# Autodesk Inventor assembly: Frame
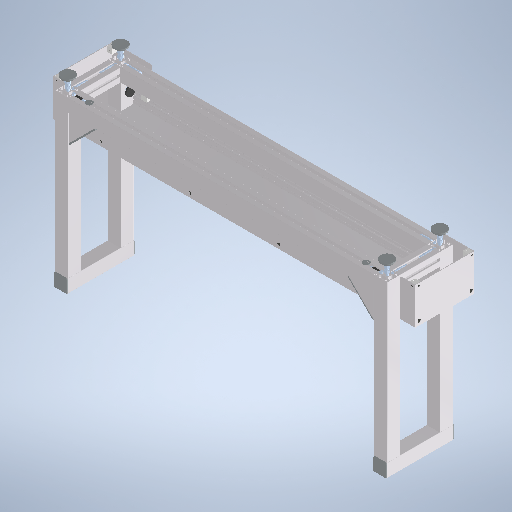
[picture p0: Inventor's stored thumbnail of the model, 512x512]
Saved by Autodesk Inventor 2025 (Build 290162010, 162A)
## iProperties
Created: 2025-01-18
Part Number: Frame
Document SubType Name: Assembly
Designer: Admin
Mass: 13411.7 g
Surface Area: 37015.5 cm^2
Volume: 4609.9 cm^3
Density: 2.90933 g/cm^3
Author: Admin
## Documents named in this file (34)
- C:\Users\Admin\GIT\HDVKBM\CAD\Krandemonstrator\Frame.iam
- C:\Users\Admin\GIT\HDVKBM\CAD\Krandemonstrator\item_61193_profil-x-8-40x40-2no180-_930_high\item_61193_profil-x-8-40x40-2no180-_930_high.ipt
- C:\Users\Admin\GIT\HDVKBM\CAD\Krandemonstrator\item_49291_profil-x-8-40x40-leicht-_120_high\item_49291_profil-x-8-40x40-leicht-_120_high.ipt
- C:\Users\Admin\GIT\HDVKBM\CAD\Krandemonstrator\item_49288_profil-x-8-40x40-4no-lei_200_high\item_49288_profil-x-8-40x40-4no-lei_200_high.ipt
- C:\Users\Admin\GIT\HDVKBM\CAD\Krandemonstrator\item_49288_profil-x-8-40x40-4no-lei_475_high\item_49288_profil-x-8-40x40-4no-lei_475_high.ipt
- C:\Users\Admin\GIT\HDVKBM\CAD\Krandemonstrator\item_67284_automatik-verbindungssat__high\item_67284_automatik-verbindungssat__high.ipt
- C:\Users\Admin\GIT\HDVKBM\CAD\Krandemonstrator\item_63697_stellfuss-d40-m8x60-grau_35_0_high\item_63697_stellfuss-d40-m8x60-grau_35_0_high.ipt
- C:\Users\Admin\GIT\HDVKBM\CAD\Krandemonstrator\item_62716_abdeckkappe-8-40x40-grau__high\item_62716_abdeckkappe-8-40x40-grau__high.ipt
- C:\Users\Admin\GIT\HDVKBM\CAD\Krandemonstrator\item_48996_automatik-verbindungssat__high\item_48996_automatik-verbindungssat__high.ipt
- C:\Users\Admin\GIT\HDVKBM\CAD\Krandemonstrator\item_41123_winkel-8-80x80-zn-weissa__high\item_41123_winkel-8-80x80-zn-weissa__high.ipt
- C:\Users\Admin\GIT\HDVKBM\CAD\Krandemonstrator\item_2618_nutenstein-8-st-m8-verzi__high\item_2618_nutenstein-8-st-m8-verzi__high.ipt
- C:\Users\Admin\GIT\HDVKBM\CAD\Krandemonstrator\item_62758_winkel-abdeckkappe-8-80x__high\item_62758_winkel-abdeckkappe-8-80x__high.ipt
- C:\Users\Admin\GIT\HDVKBM\CAD\Krandemonstrator\item_43452_stellfuss-d30-m6x45-schw_20_0_high\item_43452_stellfuss-d30-m6x45-schw_20_0_high.ipt
- C:\Users\Admin\GIT\HDVKBM\CAD\Krandemonstrator\item_2623_nutenstein-8-st-m6-verzi__high\item_2623_nutenstein-8-st-m6-verzi__high.ipt
- C:\Users\Admin\GIT\HDVKBM\CAD\Krandemonstrator\item_42005_nutenstein-8-st-m5-verzi__high\item_42005_nutenstein-8-st-m5-verzi__high.ipt
- C:\Users\Admin\GIT\HDVKBM\CAD\Krandemonstrator\item_67777_winkel-5-20-weissalumini__high\item_67777_winkel-5-20-weissalumini__high.ipt
- C:\Users\Admin\GIT\HDVKBM\CAD\Krandemonstrator\item_68092_befestigungssatz-5-2-4mm_2_high\item_68092_befestigungssatz-5-2-4mm_2_high.ipt
- C:\Users\Admin\GIT\HDVKBM\CAD\Krandemonstrator\item_47308_blech-al-2mm-naturfarben_1100_180_high\item_47308_blech-al-2mm-naturfarben_1100_180_high.ipt
- C:\Users\Admin\GIT\HDVKBM\CAD\Krandemonstrator\item_37006_nutenstein-5-st-m4-verzi__high\item_37006_nutenstein-5-st-m4-verzi__high.ipt
- C:\Users\Admin\GIT\HDVKBM\CAD\Krandemonstrator\item_47308_blech-al-2mm-naturfarben_110_1100_high\item_47308_blech-al-2mm-naturfarben_110_1100_high.ipt
- C:\Users\Admin\GIT\HDVKBM\CAD\Krandemonstrator\item_37003_profil-5-20x20-natur-370_1096_high\item_37003_profil-5-20x20-natur-370_1096_high.ipt
- C:\Users\Admin\GIT\HDVKBM\CAD\Krandemonstrator\item_43774_profil-5-20x20-1n-natur-_1096_high\item_43774_profil-5-20x20-1n-natur-_1096_high.ipt
- C:\Users\Admin\GIT\HDVKBM\CAD\Krandemonstrator\item_47308_blech-al-2mm-naturfarben_178_110_high\item_47308_blech-al-2mm-naturfarben_178_110_high.ipt
- C:\Users\Admin\GIT\HDVKBM\CAD\Krandemonstrator\item_47308_blech-al-2mm-naturfarben_120_90_high\item_47308_blech-al-2mm-naturfarben_120_90_high.ipt
- C:\Users\Admin\GIT\HDVKBM\CAD\Krandemonstrator\Frameblock.ipt
- C:\Users\Admin\GIT\HDVKBM\CAD\Krandemonstrator\item_47308_blech-al-2mm-naturfarben_120_90_high\item_47308_blech-al-2mm-naturfarben_120_90_highLH.ipt
- C:\Users\Admin\GIT\HDVKBM\CAD\Krandemonstrator\item_61196_profil-x-8-40x40-3no-lei_930_high\item_61196_profil-x-8-40x40-3no-lei_930_high.ipt
- C:\Users\Admin\Documents\Inventor\Content Center Files\R2025\de-DE\ISO 10642(2)\ISO 10642  - M3  x  8.ipt
- C:\Users\Admin\Documents\Inventor\Content Center Files\R2025\de-DE\ISO 10642(2)\ISO 10642  - M4  x  20.ipt
- C:\Users\Admin\Documents\Inventor\Content Center Files\R2025\de-DE\ISO 10642(2)\ISO 10642  - M4  x  8.ipt
- C:\Users\Admin\Documents\Inventor\Content Center Files\R2025\de-DE\ISO 10642(2)\ISO 10642  - M5  x  10.ipt
- C:\Users\Admin\Documents\Inventor\Content Center Files\R2025\de-DE\ISO 10642(2)\ISO 10642  - M5  x  12.ipt
- C:\Users\Admin\Documents\Inventor\Content Center Files\R2025\de-DE\ISO 10642(2)\ISO 10642  - M5  x  16.ipt
- C:\Users\Admin\Documents\Inventor\Content Center Files\R2025\de-DE\ISO 4762(1)\DIN EN ISO 4762 - M8 x 16.ipt
## Components (126 placed, 33 different names)
1. item_61193_profil-x-8-40x40-2no180-_930_high:1 — Starr:12, Starr:13, Starr:14
2. item_61196_profil-x-8-40x40-3no-lei_930_high:1 — Starr:17, Starr:27, Planar:1, Planar:2, Starr:47, Starr:48, Planar:68, Verschiebbar:70
3. item_49291_profil-x-8-40x40-leicht-_120_high:1 — Starr:7, Starr:8, Starr:9
4. item_49291_profil-x-8-40x40-leicht-_120_high:2 — Starr:24, Starr:25, Starr:26
5. item_49288_profil-x-8-40x40-4no-lei_200_high:1 — Starr:18, Starr:19, Starr:21, Starr:23
6. item_49288_profil-x-8-40x40-4no-lei_200_high:2 — Starr:2, Starr:4, Starr:5, Starr:6
7. item_49288_profil-x-8-40x40-4no-lei_475_high:1 — Starr:20, Starr:21, Starr:28, Starr:41, Verschiebbar:6
8. item_49288_profil-x-8-40x40-4no-lei_475_high:2 — Starr:22, Starr:23, Starr:25, Starr:27, Starr:29, Verschiebbar:2, Verschiebbar:4
9. item_49288_profil-x-8-40x40-4no-lei_475_high:3 — Starr:3, Starr:4, Starr:11, Starr:17, Verschiebbar:1, Verschiebbar:3, Planar:71
10. item_49288_profil-x-8-40x40-4no-lei_475_high:4 — Starr:1, Starr:2, Starr:9, Starr:10, Starr:14, Starr:43, Verschiebbar:5
11. item_67284_automatik-verbindungssat__high:1 — Starr:1
12. item_67284_automatik-verbindungssat__high:2 — Starr:20
13. item_67284_automatik-verbindungssat__high:3 — Starr:3
14. item_67284_automatik-verbindungssat__high:11 — Starr:22
15. item_67284_automatik-verbindungssat__high:4 — Starr:24
16. item_67284_automatik-verbindungssat__high:12 — Starr:26
17. item_67284_automatik-verbindungssat__high:5 — Starr:12
18. item_67284_automatik-verbindungssat__high:6 — Starr:13
19. item_67284_automatik-verbindungssat__high:7 — Starr:8
20. item_67284_automatik-verbindungssat__high:8 — Starr:7
21. item_48996_automatik-verbindungssat__high:1 — Starr:47
22. item_48996_automatik-verbindungssat__high:2 — Starr:48
23. item_63697_stellfuss-d40-m8x60-grau_35_0_high:1 — Starr:10
24. item_63697_stellfuss-d40-m8x60-grau_35_0_high:2 — Starr:11
25. item_63697_stellfuss-d40-m8x60-grau_35_0_high:3 — Starr:28
26. item_63697_stellfuss-d40-m8x60-grau_35_0_high:4 — Starr:29
27. item_62716_abdeckkappe-8-40x40-grau__high:1 — Starr:5
28. item_62716_abdeckkappe-8-40x40-grau__high:2 — Starr:6
29. item_62716_abdeckkappe-8-40x40-grau__high:3 — Starr:18
30. item_62716_abdeckkappe-8-40x40-grau__high:4 — Starr:19
31. item_41123_winkel-8-80x80-zn-weissa__high:1 — Verschiebbar:2, Planar:2, Starr:38
32. item_41123_winkel-8-80x80-zn-weissa__high:2 — Verschiebbar:1, Planar:1, Starr:39
33. item_2618_nutenstein-8-st-m8-verzi__high:5
34. item_2618_nutenstein-8-st-m8-verzi__high:3
35. item_2618_nutenstein-8-st-m8-verzi__high:2
36. item_2618_nutenstein-8-st-m8-verzi__high:6
37. item_2618_nutenstein-8-st-m8-verzi__high:4
38. item_2618_nutenstein-8-st-m8-verzi__high:8
39. item_2618_nutenstein-8-st-m8-verzi__high:1
40. item_2618_nutenstein-8-st-m8-verzi__high:7
41. DIN EN ISO 4762 M8 x 16:1
42. DIN EN ISO 4762 M8 x 16:2
43. DIN EN ISO 4762 M8 x 16:3
44. DIN EN ISO 4762 M8 x 16:4
45. DIN EN ISO 4762 M8 x 16:5
46. DIN EN ISO 4762 M8 x 16:6
47. DIN EN ISO 4762 M8 x 16:7
48. DIN EN ISO 4762 M8 x 16:8
49. item_62758_winkel-abdeckkappe-8-80x__high:1 — Starr:38
50. item_62758_winkel-abdeckkappe-8-80x__high:2 — Starr:39
51. item_2623_nutenstein-8-st-m6-verzi__high:2 — Starr:42, Starr:43
52. item_2623_nutenstein-8-st-m6-verzi__high:1 — Starr:40, Starr:41
53. item_43452_stellfuss-d30-m6x45-schw_20_0_high:1 — Starr:40
54. item_43452_stellfuss-d30-m6x45-schw_20_0_high:2 — Starr:42
55. Frameblock:1 — Starr:73, Starr:84
56. Frameblock:2 — Starr:74, Starr:83
57. Frameblock:3 — Starr:75
58. Frameblock:4 — Starr:76, Starr:82
59. Frameblock:5 — Starr:78
60. Frameblock:6 — Starr:77, Starr:81
61. Frameblock:7 — Starr:79
62. Frameblock:8 — Starr:80
63. item_37006_nutenstein-5-st-m4-verzi__high:1 — Starr:61
64. item_37006_nutenstein-5-st-m4-verzi__high:2 — Starr:63
65. item_37006_nutenstein-5-st-m4-verzi__high:3 — Starr:62
66. item_37006_nutenstein-5-st-m4-verzi__high:4 — Starr:60
67. item_37006_nutenstein-5-st-m4-verzi__high:5 — Starr:81
68. item_37006_nutenstein-5-st-m4-verzi__high:6 — Starr:84
69. item_37006_nutenstein-5-st-m4-verzi__high:7 — Starr:82
70. item_37006_nutenstein-5-st-m4-verzi__high:8 — Starr:83
71. item_37006_nutenstein-5-st-m4-verzi__high:9
72. item_37006_nutenstein-5-st-m4-verzi__high:10
73. item_37006_nutenstein-5-st-m4-verzi__high:11
74. item_37006_nutenstein-5-st-m4-verzi__high:12
75. item_42005_nutenstein-8-st-m5-verzi__high:1 — Starr:45
76. item_42005_nutenstein-8-st-m5-verzi__high:2 — Starr:44
77. item_42005_nutenstein-8-st-m5-verzi__high:3 — Starr:52
78. item_42005_nutenstein-8-st-m5-verzi__high:4 — Starr:53
79. item_43774_profil-5-20x20-1n-natur-_1096_high:1 — Planar:73, Planar:76
80. item_37003_profil-5-20x20-natur-370_1096_high:1
81. item_47308_blech-al-2mm-naturfarben_110_1100_high:1 — Starr:64, Starr:65, Starr:66, Starr:67, Planar:71, Starr:68, Verschiebbar:70, Starr:69, Starr:70
82. item_47308_blech-al-2mm-naturfarben_178_110_high:1 — Starr:69, Starr:71, Starr:80
83. item_47308_blech-al-2mm-naturfarben_178_110_high:2 — Starr:70, Starr:72, Starr:79
84. item_47308_blech-al-2mm-naturfarben_120_90_highLH:1 — Starr:72, Starr:76, Starr:77, Starr:78
85. item_47308_blech-al-2mm-naturfarben_120_90_high:2 — Starr:71, Starr:73, Starr:74, Starr:75
86. item_47308_blech-al-2mm-naturfarben_1100_180_high:1 — Planar:68, Starr:68, Planar:76
87. item_67777_winkel-5-20-weissalumini__high:1 — Starr:44, Starr:49, Verschiebbar:6, Planar:73
88. item_67777_winkel-5-20-weissalumini__high:2 — Starr:45, Starr:46, Verschiebbar:5
89. item_67777_winkel-5-20-weissalumini__high:3 — Starr:50, Starr:53, Verschiebbar:4
90. item_67777_winkel-5-20-weissalumini__high:4 — Starr:51, Starr:52, Verschiebbar:3
91. item_68092_befestigungssatz-5-2-4mm_2_high:1 — Starr:49
92. item_68092_befestigungssatz-5-2-4mm_2_high:2 — Starr:46
93. item_68092_befestigungssatz-5-2-4mm_2_high:3 — Starr:50
94. item_68092_befestigungssatz-5-2-4mm_2_high:4 — Starr:51
95. DIN EN ISO 10642 M3  x  8:1
96. DIN EN ISO 10642 M3  x  8:2
97. DIN EN ISO 10642 M3  x  8:3
98. DIN EN ISO 10642 M4  x  20:1
99. DIN EN ISO 10642 M3  x  8:4
100. DIN EN ISO 10642 M3  x  8:5
101. DIN EN ISO 10642 M3  x  8:6
102. DIN EN ISO 10642 M4  x  20:2
103. DIN EN ISO 10642 M3  x  8:7
104. DIN EN ISO 10642 M3  x  8:8
105. DIN EN ISO 10642 M3  x  8:9
106. DIN EN ISO 10642 M3  x  8:10
107. DIN EN ISO 10642 M3  x  8:11
108. DIN EN ISO 10642 M3  x  8:12
109. DIN EN ISO 10642 M4  x  20:3
110. DIN EN ISO 10642 M4  x  20:4
111. DIN EN ISO 10642 M4  x  8:1
112. DIN EN ISO 10642 M4  x  8:2
113. DIN EN ISO 10642 M4  x  8:3
114. DIN EN ISO 10642 M4  x  8:4
115. DIN EN ISO 10642 M5  x  10:1
116. DIN EN ISO 10642 M5  x  10:2
117. DIN EN ISO 10642 M5  x  10:3
118. DIN EN ISO 10642 M5  x  10:4
119. DIN EN ISO 10642 M4  x  8:5 — Starr:60, Starr:67
120. DIN EN ISO 10642 M4  x  8:6 — Starr:62, Starr:64
121. DIN EN ISO 10642 M4  x  8:7 — Starr:61, Starr:66
122. DIN EN ISO 10642 M4  x  8:8 — Starr:63, Starr:65
123. DIN EN ISO 10642 M5  x  12:1
124. DIN EN ISO 10642 M5  x  12:2
125. DIN EN ISO 10642 M5  x  16:1
126. DIN EN ISO 10642 M5  x  16:2
## Relationships (138: WeldJoint 84, Mate 24, PlanarJoint 14, Insert 8, TranslationJoint 8)
- Starr:1 [WeldJoint]: item_49288_profil-x-8-40x40-4no-lei_475_high:4 ↔ item_67284_automatik-verbindungssat__high:1
- Starr:2 [WeldJoint]: item_49288_profil-x-8-40x40-4no-lei_200_high:2 ↔ item_49288_profil-x-8-40x40-4no-lei_475_high:4
- Starr:3 [WeldJoint]: item_49288_profil-x-8-40x40-4no-lei_475_high:3 ↔ item_67284_automatik-verbindungssat__high:3
- Starr:4 [WeldJoint]: item_49288_profil-x-8-40x40-4no-lei_200_high:2 ↔ item_49288_profil-x-8-40x40-4no-lei_475_high:3
- Starr:5 [WeldJoint]: item_49288_profil-x-8-40x40-4no-lei_200_high:2 ↔ item_62716_abdeckkappe-8-40x40-grau__high:1
- Starr:6 [WeldJoint]: item_49288_profil-x-8-40x40-4no-lei_200_high:2 ↔ item_62716_abdeckkappe-8-40x40-grau__high:2
- Starr:7 [WeldJoint]: item_49291_profil-x-8-40x40-leicht-_120_high:1 ↔ item_67284_automatik-verbindungssat__high:8
- Starr:8 [WeldJoint]: item_49291_profil-x-8-40x40-leicht-_120_high:1 ↔ item_67284_automatik-verbindungssat__high:7
- Starr:9 [WeldJoint]: item_49291_profil-x-8-40x40-leicht-_120_high:1 ↔ item_49288_profil-x-8-40x40-4no-lei_475_high:4
- Starr:10 [WeldJoint]: item_49288_profil-x-8-40x40-4no-lei_475_high:4 ↔ item_63697_stellfuss-d40-m8x60-grau_35_0_high:1
- Starr:11 [WeldJoint]: item_49288_profil-x-8-40x40-4no-lei_475_high:3 ↔ item_63697_stellfuss-d40-m8x60-grau_35_0_high:2
- Starr:12 [WeldJoint]: item_61193_profil-x-8-40x40-2no180-_930_high:1 ↔ item_67284_automatik-verbindungssat__high:5
- Starr:13 [WeldJoint]: item_61193_profil-x-8-40x40-2no180-_930_high:1 ↔ item_67284_automatik-verbindungssat__high:6
- Starr:14 [WeldJoint]: item_61193_profil-x-8-40x40-2no180-_930_high:1 ↔ item_49288_profil-x-8-40x40-4no-lei_475_high:4
- Starr:17 [WeldJoint]: item_61196_profil-x-8-40x40-3no-lei_930_high:1 ↔ item_49288_profil-x-8-40x40-4no-lei_475_high:3
- Starr:18 [WeldJoint]: item_49288_profil-x-8-40x40-4no-lei_200_high:1 ↔ item_62716_abdeckkappe-8-40x40-grau__high:3
- Starr:19 [WeldJoint]: item_49288_profil-x-8-40x40-4no-lei_200_high:1 ↔ item_62716_abdeckkappe-8-40x40-grau__high:4
- Starr:20 [WeldJoint]: item_49288_profil-x-8-40x40-4no-lei_475_high:1 ↔ item_67284_automatik-verbindungssat__high:2
- Starr:21 [WeldJoint]: item_49288_profil-x-8-40x40-4no-lei_200_high:1 ↔ item_49288_profil-x-8-40x40-4no-lei_475_high:1
- Starr:22 [WeldJoint]: item_49288_profil-x-8-40x40-4no-lei_475_high:2 ↔ item_67284_automatik-verbindungssat__high:11
- Starr:23 [WeldJoint]: item_49288_profil-x-8-40x40-4no-lei_200_high:1 ↔ item_49288_profil-x-8-40x40-4no-lei_475_high:2
- Starr:24 [WeldJoint]: item_49291_profil-x-8-40x40-leicht-_120_high:2 ↔ item_67284_automatik-verbindungssat__high:4
- Starr:25 [WeldJoint]: item_49291_profil-x-8-40x40-leicht-_120_high:2 ↔ item_49288_profil-x-8-40x40-4no-lei_475_high:2
- Starr:26 [WeldJoint]: item_49291_profil-x-8-40x40-leicht-_120_high:2 ↔ item_67284_automatik-verbindungssat__high:12
- Starr:27 [WeldJoint]: item_61196_profil-x-8-40x40-3no-lei_930_high:1 ↔ item_49288_profil-x-8-40x40-4no-lei_475_high:2
- Starr:28 [WeldJoint]: item_49288_profil-x-8-40x40-4no-lei_475_high:1 ↔ item_63697_stellfuss-d40-m8x60-grau_35_0_high:3
- Starr:29 [WeldJoint]: item_49288_profil-x-8-40x40-4no-lei_475_high:2 ↔ item_63697_stellfuss-d40-m8x60-grau_35_0_high:4
- [Insert]: item_41123_winkel-8-80x80-zn-weissa__high:2 ↔ DIN EN ISO 4762 M8 x 16:1
- [Insert]: item_41123_winkel-8-80x80-zn-weissa__high:2 ↔ DIN EN ISO 4762 M8 x 16:2
- [Insert]: item_41123_winkel-8-80x80-zn-weissa__high:1 ↔ DIN EN ISO 4762 M8 x 16:3
- [Insert]: item_41123_winkel-8-80x80-zn-weissa__high:1 ↔ DIN EN ISO 4762 M8 x 16:4
- [Insert]: item_41123_winkel-8-80x80-zn-weissa__high:2 ↔ DIN EN ISO 4762 M8 x 16:5
- [Insert]: item_41123_winkel-8-80x80-zn-weissa__high:2 ↔ DIN EN ISO 4762 M8 x 16:6
- [Insert]: item_41123_winkel-8-80x80-zn-weissa__high:1 ↔ DIN EN ISO 4762 M8 x 16:7
- [Insert]: item_41123_winkel-8-80x80-zn-weissa__high:1 ↔ DIN EN ISO 4762 M8 x 16:8
- [WeldJoint]: item_2618_nutenstein-8-st-m8-verzi__high:6 ↔ DIN EN ISO 4762 M8 x 16:6
- [WeldJoint]: item_2618_nutenstein-8-st-m8-verzi__high:2 ↔ DIN EN ISO 4762 M8 x 16:5
- [WeldJoint]: item_2618_nutenstein-8-st-m8-verzi__high:4 ↔ DIN EN ISO 4762 M8 x 16:8
- [WeldJoint]: item_2618_nutenstein-8-st-m8-verzi__high:8 ↔ DIN EN ISO 4762 M8 x 16:7
- [WeldJoint]: item_2618_nutenstein-8-st-m8-verzi__high:1 ↔ DIN EN ISO 4762 M8 x 16:4
- [WeldJoint]: item_2618_nutenstein-8-st-m8-verzi__high:7 ↔ DIN EN ISO 4762 M8 x 16:3
- [WeldJoint]: item_2618_nutenstein-8-st-m8-verzi__high:3 ↔ DIN EN ISO 4762 M8 x 16:2
- [WeldJoint]: item_2618_nutenstein-8-st-m8-verzi__high:5 ↔ DIN EN ISO 4762 M8 x 16:1
- Verschiebbar:1 [TranslationJoint]: item_49288_profil-x-8-40x40-4no-lei_475_high:3 ↔ item_41123_winkel-8-80x80-zn-weissa__high:2
- Planar:1: item_61196_profil-x-8-40x40-3no-lei_930_high:1 ↔ item_41123_winkel-8-80x80-zn-weissa__high:2
- Verschiebbar:2 [TranslationJoint]: item_49288_profil-x-8-40x40-4no-lei_475_high:2 ↔ item_41123_winkel-8-80x80-zn-weissa__high:1
- Planar:2: item_61196_profil-x-8-40x40-3no-lei_930_high:1 ↔ item_41123_winkel-8-80x80-zn-weissa__high:1
- Starr:38 [WeldJoint]: item_41123_winkel-8-80x80-zn-weissa__high:1 ↔ item_62758_winkel-abdeckkappe-8-80x__high:1
- Starr:39 [WeldJoint]: item_41123_winkel-8-80x80-zn-weissa__high:2 ↔ item_62758_winkel-abdeckkappe-8-80x__high:2
- Starr:40 [WeldJoint]: item_2623_nutenstein-8-st-m6-verzi__high:1 ↔ item_43452_stellfuss-d30-m6x45-schw_20_0_high:1
- Starr:41 [WeldJoint] (-60 mm): item_49288_profil-x-8-40x40-4no-lei_475_high:1 ↔ item_2623_nutenstein-8-st-m6-verzi__high:1
- Starr:42 [WeldJoint]: item_2623_nutenstein-8-st-m6-verzi__high:2 ↔ item_43452_stellfuss-d30-m6x45-schw_20_0_high:2
- Starr:43 [WeldJoint] (-60 mm): item_49288_profil-x-8-40x40-4no-lei_475_high:4 ↔ item_2623_nutenstein-8-st-m6-verzi__high:2
- Starr:44 [WeldJoint] (-5 mm): item_42005_nutenstein-8-st-m5-verzi__high:2 ↔ item_67777_winkel-5-20-weissalumini__high:1
- Starr:45 [WeldJoint] (-5 mm): item_42005_nutenstein-8-st-m5-verzi__high:1 ↔ item_67777_winkel-5-20-weissalumini__high:2
- Starr:46 [WeldJoint]: item_67777_winkel-5-20-weissalumini__high:2 ↔ item_68092_befestigungssatz-5-2-4mm_2_high:2
- Starr:47 [WeldJoint]: item_61196_profil-x-8-40x40-3no-lei_930_high:1 ↔ item_48996_automatik-verbindungssat__high:1
- Starr:48 [WeldJoint]: item_61196_profil-x-8-40x40-3no-lei_930_high:1 ↔ item_48996_automatik-verbindungssat__high:2
- Starr:49 [WeldJoint]: item_67777_winkel-5-20-weissalumini__high:1 ↔ item_68092_befestigungssatz-5-2-4mm_2_high:1
- [Mate]: item_67777_winkel-5-20-weissalumini__high:1 ↔ DIN EN ISO 10642 M5  x  12:1
- [Mate]: item_67777_winkel-5-20-weissalumini__high:2 ↔ DIN EN ISO 10642 M5  x  12:2
- Starr:50 [WeldJoint]: item_67777_winkel-5-20-weissalumini__high:3 ↔ item_68092_befestigungssatz-5-2-4mm_2_high:3
- Starr:51 [WeldJoint]: item_67777_winkel-5-20-weissalumini__high:4 ↔ item_68092_befestigungssatz-5-2-4mm_2_high:4
- [Mate]: item_67777_winkel-5-20-weissalumini__high:3 ↔ DIN EN ISO 10642 M5  x  16:1
- [Mate]: item_67777_winkel-5-20-weissalumini__high:4 ↔ DIN EN ISO 10642 M5  x  16:2
- Starr:52 [WeldJoint] (-5 mm): item_42005_nutenstein-8-st-m5-verzi__high:3 ↔ item_67777_winkel-5-20-weissalumini__high:4
- Starr:53 [WeldJoint] (-5 mm): item_42005_nutenstein-8-st-m5-verzi__high:4 ↔ item_67777_winkel-5-20-weissalumini__high:3
- Verschiebbar:3 [TranslationJoint] (2 mm): item_49288_profil-x-8-40x40-4no-lei_475_high:3 ↔ item_67777_winkel-5-20-weissalumini__high:4
- Verschiebbar:4 [TranslationJoint]: item_49288_profil-x-8-40x40-4no-lei_475_high:2 ↔ item_67777_winkel-5-20-weissalumini__high:3
- [PlanarJoint]: item_37003_profil-5-20x20-natur-370_1096_high:1 ↔ item_67777_winkel-5-20-weissalumini__high:4
- [PlanarJoint]: item_37003_profil-5-20x20-natur-370_1096_high:1 ↔ item_67777_winkel-5-20-weissalumini__high:3
- Verschiebbar:5 [TranslationJoint]: item_49288_profil-x-8-40x40-4no-lei_475_high:4 ↔ item_67777_winkel-5-20-weissalumini__high:2
- Verschiebbar:6 [TranslationJoint]: item_49288_profil-x-8-40x40-4no-lei_475_high:1 ↔ item_67777_winkel-5-20-weissalumini__high:1
- [PlanarJoint]: item_37003_profil-5-20x20-natur-370_1096_high:1 ↔ item_47308_blech-al-2mm-naturfarben_1100_180_high:1
- Starr:60 [WeldJoint]: item_37006_nutenstein-5-st-m4-verzi__high:4 ↔ DIN EN ISO 10642 M4  x  8:5
- Starr:61 [WeldJoint]: item_37006_nutenstein-5-st-m4-verzi__high:1 ↔ DIN EN ISO 10642 M4  x  8:7
- Starr:62 [WeldJoint]: item_37006_nutenstein-5-st-m4-verzi__high:3 ↔ DIN EN ISO 10642 M4  x  8:6
- Starr:63 [WeldJoint]: item_37006_nutenstein-5-st-m4-verzi__high:2 ↔ DIN EN ISO 10642 M4  x  8:8
- Planar:68 (75 mm): item_61196_profil-x-8-40x40-3no-lei_930_high:1 ↔ item_47308_blech-al-2mm-naturfarben_1100_180_high:1
- Starr:64 [WeldJoint]: item_47308_blech-al-2mm-naturfarben_110_1100_high:1 ↔ DIN EN ISO 10642 M4  x  8:6
- Starr:65 [WeldJoint]: item_47308_blech-al-2mm-naturfarben_110_1100_high:1 ↔ DIN EN ISO 10642 M4  x  8:8
- Starr:66 [WeldJoint]: item_47308_blech-al-2mm-naturfarben_110_1100_high:1 ↔ DIN EN ISO 10642 M4  x  8:7
- Starr:67 [WeldJoint]: item_47308_blech-al-2mm-naturfarben_110_1100_high:1 ↔ DIN EN ISO 10642 M4  x  8:5
- [PlanarJoint]: item_37003_profil-5-20x20-natur-370_1096_high:1 ↔ item_47308_blech-al-2mm-naturfarben_110_1100_high:1
- [PlanarJoint]: item_37003_profil-5-20x20-natur-370_1096_high:1 ↔ item_47308_blech-al-2mm-naturfarben_110_1100_high:1
- [TranslationJoint]: item_37003_profil-5-20x20-natur-370_1096_high:1 ↔ item_47308_blech-al-2mm-naturfarben_110_1100_high:1
- Planar:71: item_49288_profil-x-8-40x40-4no-lei_475_high:3 ↔ item_47308_blech-al-2mm-naturfarben_110_1100_high:1
- Starr:68 [WeldJoint]: item_47308_blech-al-2mm-naturfarben_110_1100_high:1 ↔ item_47308_blech-al-2mm-naturfarben_1100_180_high:1
- Verschiebbar:70 [TranslationJoint]: item_61196_profil-x-8-40x40-3no-lei_930_high:1 ↔ item_47308_blech-al-2mm-naturfarben_110_1100_high:1
- [PlanarJoint]: item_43774_profil-5-20x20-1n-natur-_1096_high:1 ↔ item_47308_blech-al-2mm-naturfarben_1100_180_high:1
- Planar:73: item_43774_profil-5-20x20-1n-natur-_1096_high:1 ↔ item_67777_winkel-5-20-weissalumini__high:1
- [PlanarJoint]: item_43774_profil-5-20x20-1n-natur-_1096_high:1 ↔ item_67777_winkel-5-20-weissalumini__high:2
- [PlanarJoint]: item_49288_profil-x-8-40x40-4no-lei_475_high:4 ↔ item_43774_profil-5-20x20-1n-natur-_1096_high:1
- Planar:76 (-2 mm): item_43774_profil-5-20x20-1n-natur-_1096_high:1 ↔ item_47308_blech-al-2mm-naturfarben_1100_180_high:1
- Starr:69 [WeldJoint]: item_47308_blech-al-2mm-naturfarben_110_1100_high:1 ↔ item_47308_blech-al-2mm-naturfarben_178_110_high:1
- Starr:70 [WeldJoint]: item_47308_blech-al-2mm-naturfarben_110_1100_high:1 ↔ item_47308_blech-al-2mm-naturfarben_178_110_high:2
- Starr:71 [WeldJoint]: item_47308_blech-al-2mm-naturfarben_178_110_high:1 ↔ item_47308_blech-al-2mm-naturfarben_120_90_high:2
- Starr:72 [WeldJoint]: item_47308_blech-al-2mm-naturfarben_178_110_high:2 ↔ item_47308_blech-al-2mm-naturfarben_120_90_highLH:1
- [Mate]: item_47308_blech-al-2mm-naturfarben_178_110_high:1 ↔ DIN EN ISO 10642 M5  x  10:1
- [Mate]: item_47308_blech-al-2mm-naturfarben_178_110_high:1 ↔ DIN EN ISO 10642 M5  x  10:2
- [Mate]: item_47308_blech-al-2mm-naturfarben_178_110_high:2 ↔ DIN EN ISO 10642 M5  x  10:3
- [Mate]: item_47308_blech-al-2mm-naturfarben_178_110_high:2 ↔ DIN EN ISO 10642 M5  x  10:4
- Starr:73 [WeldJoint]: Frameblock:1 ↔ item_47308_blech-al-2mm-naturfarben_120_90_high:2
- Starr:74 [WeldJoint]: Frameblock:2 ↔ item_47308_blech-al-2mm-naturfarben_120_90_high:2
- Starr:75 [WeldJoint]: Frameblock:3 ↔ item_47308_blech-al-2mm-naturfarben_120_90_high:2
- Starr:76 [WeldJoint]: Frameblock:4 ↔ item_47308_blech-al-2mm-naturfarben_120_90_highLH:1
- Starr:77 [WeldJoint]: Frameblock:6 ↔ item_47308_blech-al-2mm-naturfarben_120_90_highLH:1
- Starr:78 [WeldJoint]: Frameblock:5 ↔ item_47308_blech-al-2mm-naturfarben_120_90_highLH:1
- Starr:79 [WeldJoint]: Frameblock:7 ↔ item_47308_blech-al-2mm-naturfarben_178_110_high:2
- Starr:80 [WeldJoint]: Frameblock:8 ↔ item_47308_blech-al-2mm-naturfarben_178_110_high:1
- [Mate]: item_47308_blech-al-2mm-naturfarben_110_1100_high:1 ↔ DIN EN ISO 10642 M3  x  8:4
- [Mate]: item_47308_blech-al-2mm-naturfarben_178_110_high:2 ↔ DIN EN ISO 10642 M3  x  8:5
- Starr:81 [WeldJoint]: Frameblock:6 ↔ item_37006_nutenstein-5-st-m4-verzi__high:5
- [Mate]: Frameblock:6 ↔ DIN EN ISO 10642 M4  x  20:1
- [Mate]: item_47308_blech-al-2mm-naturfarben_178_110_high:2 ↔ DIN EN ISO 10642 M3  x  8:2
- [Mate]: item_47308_blech-al-2mm-naturfarben_120_90_highLH:1 ↔ DIN EN ISO 10642 M3  x  8:3
- [Mate]: item_47308_blech-al-2mm-naturfarben_120_90_highLH:1 ↔ DIN EN ISO 10642 M3  x  8:1
- [Mate]: item_47308_blech-al-2mm-naturfarben_120_90_highLH:1 ↔ DIN EN ISO 10642 M3  x  8:6
- [Mate]: Frameblock:4 ↔ DIN EN ISO 10642 M4  x  20:2
- Starr:82 [WeldJoint]: Frameblock:4 ↔ item_37006_nutenstein-5-st-m4-verzi__high:7
- [Mate]: item_47308_blech-al-2mm-naturfarben_120_90_high:2 ↔ DIN EN ISO 10642 M3  x  8:7
- [Mate]: item_47308_blech-al-2mm-naturfarben_120_90_high:2 ↔ DIN EN ISO 10642 M3  x  8:8
- [Mate]: item_47308_blech-al-2mm-naturfarben_120_90_high:2 ↔ DIN EN ISO 10642 M3  x  8:9
- [Mate]: item_47308_blech-al-2mm-naturfarben_178_110_high:1 ↔ DIN EN ISO 10642 M3  x  8:10
- [Mate]: item_47308_blech-al-2mm-naturfarben_178_110_high:1 ↔ DIN EN ISO 10642 M3  x  8:11
- [Mate]: item_47308_blech-al-2mm-naturfarben_110_1100_high:1 ↔ DIN EN ISO 10642 M3  x  8:12
- Starr:83 [WeldJoint]: Frameblock:2 ↔ item_37006_nutenstein-5-st-m4-verzi__high:8
- [Mate]: Frameblock:2 ↔ DIN EN ISO 10642 M4  x  20:3
- Starr:84 [WeldJoint]: Frameblock:1 ↔ item_37006_nutenstein-5-st-m4-verzi__high:6
- [Mate]: Frameblock:1 ↔ DIN EN ISO 10642 M4  x  20:4
- [WeldJoint]: item_47308_blech-al-2mm-naturfarben_1100_180_high:1 ↔ DIN EN ISO 10642 M4  x  8:1
- [WeldJoint]: item_47308_blech-al-2mm-naturfarben_1100_180_high:1 ↔ DIN EN ISO 10642 M4  x  8:2
- [WeldJoint]: item_47308_blech-al-2mm-naturfarben_1100_180_high:1 ↔ DIN EN ISO 10642 M4  x  8:3
- [WeldJoint]: item_47308_blech-al-2mm-naturfarben_1100_180_high:1 ↔ DIN EN ISO 10642 M4  x  8:4
- [WeldJoint]: item_37006_nutenstein-5-st-m4-verzi__high:12 ↔ DIN EN ISO 10642 M4  x  8:3
- [WeldJoint]: item_37006_nutenstein-5-st-m4-verzi__high:11 ↔ DIN EN ISO 10642 M4  x  8:4
- [WeldJoint]: item_37006_nutenstein-5-st-m4-verzi__high:9 ↔ DIN EN ISO 10642 M4  x  8:1
- [WeldJoint]: item_37006_nutenstein-5-st-m4-verzi__high:10 ↔ DIN EN ISO 10642 M4  x  8:2
